# Autodesk Inventor assembly: extending arm thing
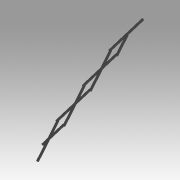
[picture p0: Inventor's stored thumbnail of the model, 180x180]
Saved by Autodesk Inventor 2016 (Build 200138000, 138)
## iProperties
Created: 2015-12-16
Part Number: extending arm thing
Document SubType Name: Assembly
Designer: Delta
Author: Delta
## Documents named in this file (4)
- C:\Robotics\CAD\2015-16\custom cad parts\extending arm thing.iam
- C:\Robotics\CAD\2015-16\COTSParts\Actobotics\585 parts\585398.ipt
- C:\Robotics\CAD\2015-16\COTSParts\Actobotics\585 parts\585392.ipt
- C:\Robotics\CAD\2015-16\COTSParts\Actobotics\585 parts\585396.ipt
## Components (8 placed, 3 different names)
1. 585398:1 — Insert:4, Insert:6, Insert:13
2. 585398:2 — Insert:3, Insert:14
3. 585398:4 — Insert:3, Insert:4, Insert:5
4. 585398:5 — Insert:6, Insert:7, Insert:15
5. 585398:6 — Insert:5, Insert:7, Insert:11
6. 585398:9 — Insert:11, Insert:16
7. 585392:1 — Insert:15, Insert:16
8. 585396:1 — Insert:13, Insert:14
## Relationships (10: Insert 10)
- Insert:3: 585398:2 ↔ 585398:4
- Insert:4: 585398:1 ↔ 585398:4
- Insert:5: 585398:4 ↔ 585398:6
- Insert:6: 585398:1 ↔ 585398:5
- Insert:7: 585398:5 ↔ 585398:6
- Insert:11: 585398:6 ↔ 585398:9
- Insert:13: 585398:1 ↔ 585396:1
- Insert:14: 585398:2 ↔ 585396:1
- Insert:15: 585398:5 ↔ 585392:1
- Insert:16: 585398:9 ↔ 585392:1
